# Autodesk Inventor assembly: GE-12078
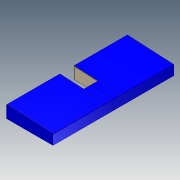
[picture p0: Inventor's stored thumbnail of the model, 180x180]
Saved by Autodesk Inventor 2012 (Build 160160000, 160)
## iProperties
Created: 2011-10-09
Part Number: GE-12078
Document SubType Name: Assembly
Designer: dfoster
Description: Fender Assembly
Title: Fender Assembly
Author: dfoster
## Documents named in this file (8)
- C:\Data Folder\FRC 2012 Field\Components\GE-12078.iam
- C:\Data Folder\FRC 2012 Field\Components\GE-12083.ipt
- C:\Data Folder\FRC 2012 Field\Components\GE-12084.ipt
- C:\Data Folder\FRC 2012 Field\Components\GE-12085.ipt
- C:\Data Folder\FRC 2012 Field\Components\GE-12103.iam
- C:\Data Folder\FRC 2012 Field\Components\GE-12103_MIR.iam
- C:\Data Folder\FRC 2012 Field\Components\GE-12078-01.ipt
- C:\Data Folder\FRC 2012 Field\Components\GE-12078-02.ipt
## Components (20 placed, 7 different names)
1. GE-12083:1 — Flush:8, Mate:12, Mate:18, Flush:17, Flush:20
2. GE-12083:2 — Flush:8, Mate:12, Flush:10, Mate:17
3. GE-12084:1 — Flush:10, Flush:15
4. GE-12084:2 — Flush:14, Mate:19, Flush:20
5. GE-12085:1 — Flush:14, Flush:16
6. GE-12085:2 — Flush:15, Flush:16, Mate:17
7. GE-12103:1 [sub-assembly] — Flush:18, Flush:19, Mate:20
8. GE-12103_MIR:1 [sub-assembly] — Mate:18, Mate:19, Flush:17, Flush:18, Flush:19, Mate:20, Mate:21, Flush:21, Flush:22, Mate:22, Flush:23, Flush:24, Flush:25, Mate:23, Flush:26, Mate:24, Mate:25, Flush:27, Flush:28, Flush:29, Flush:30, Mate:26, Flush:31, Mate:27
9. GE-12078-01:1 — Mate:21, Flush:21, Flush:22
10. GE-12078-02:1 — Mate:22, Flush:23, Flush:24
11. GE-12078-01:2 — Mate:24, Flush:27, Flush:28
12. GE-12078-01:3 — Mate:25, Flush:29, Flush:30
13. GE-12078-01:4 — Flush:25, Mate:23, Flush:26
14. GE-12078-02:2 — Mate:26, Flush:31, Mate:27
15. GE-12078-01:5
16. GE-12078-02:3
17. GE-12078-01:6
18. GE-12078-01:7
19. GE-12078-01:8
20. GE-12078-02:4
## Relationships (32: Flush 20, Mate 12)
- Flush:8: GE-12083:1 ↔ GE-12083:2
- Mate:12: GE-12083:1 ↔ GE-12083:2
- Flush:10: GE-12083:2 ↔ GE-12084:1
- Flush:14: GE-12084:2 ↔ GE-12085:1
- Flush:15: GE-12084:1 ↔ GE-12085:2
- Flush:16: GE-12085:1 ↔ GE-12085:2
- Mate:17: GE-12083:2 ↔ GE-12085:2
- Mate:18: GE-12083:1 ↔ GE-12103_MIR:1
- Mate:19: GE-12084:2 ↔ GE-12103_MIR:1
- Flush:17: GE-12083:1 ↔ GE-12103_MIR:1
- Flush:18: GE-12103:1 ↔ GE-12103_MIR:1
- Flush:19: GE-12103:1 ↔ GE-12103_MIR:1
- Mate:20: GE-12103:1 ↔ GE-12103_MIR:1
- Flush:20: GE-12083:1 ↔ GE-12084:2
- Mate:21: GE-12103_MIR:1 ↔ GE-12078-01:1
- Flush:21: GE-12103_MIR:1 ↔ GE-12078-01:1
- Flush:22: GE-12103_MIR:1 ↔ GE-12078-01:1
- Mate:22: GE-12103_MIR:1 ↔ GE-12078-02:1
- Flush:23: GE-12103_MIR:1 ↔ GE-12078-02:1
- Flush:24: GE-12103_MIR:1 ↔ GE-12078-02:1
- Flush:25: GE-12103_MIR:1 ↔ GE-12078-01:4
- Mate:23: GE-12103_MIR:1 ↔ GE-12078-01:4
- Flush:26: GE-12103_MIR:1 ↔ GE-12078-01:4
- Mate:24: GE-12103_MIR:1 ↔ GE-12078-01:2
- Mate:25: GE-12103_MIR:1 ↔ GE-12078-01:3
- Flush:27: GE-12103_MIR:1 ↔ GE-12078-01:2
- Flush:28: GE-12103_MIR:1 ↔ GE-12078-01:2
- Flush:29: GE-12103_MIR:1 ↔ GE-12078-01:3
- Flush:30: GE-12103_MIR:1 ↔ GE-12078-01:3
- Mate:26: GE-12103_MIR:1 ↔ GE-12078-02:2
- Flush:31: GE-12103_MIR:1 ↔ GE-12078-02:2
- Mate:27: GE-12103_MIR:1 ↔ GE-12078-02:2
